# Autodesk Inventor assembly: Elevator HTD Iddler Pulley
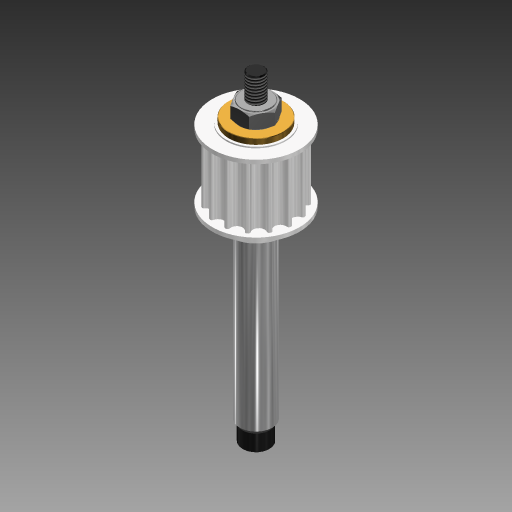
[picture p0: Inventor's stored thumbnail of the model, 512x512]
Saved by Autodesk Inventor 2023 (Build 270158030, 158C)
## iProperties
Created: 2023-02-09
Part Number: Elevator HTD Iddler Pulley
Document SubType Name: Assembly
Designer: Max Boord
Author: Max Boord
## Documents named in this file (11)
- D:\Collaborative Robots\COTS Parts\Elevators\Rev & WCP Elevator\Elevator HTD Iddler Pulley.iam
- D:\Collaborative Robots\COTS Parts\Power Transfer\Belts and Pullies\15T x 18mm Wide HTD 5mm Pulley (TTB-0058).ipt
- D:\Collaborative Robots\COTS Parts\Power Transfer\Bearings and Bushings\WCP 500 Hex Bushing.ipt
- D:\Collaborative Robots\COTS Parts\Hardware\Spacers\Spacers & Standoffs.ipt
- D:\Collaborative Robots\COTS Parts\Hardware\Fasteners\Washers.ipt
- D:\Collaborative Robots\COTS Parts\Hardware\Fasteners\Machine Screws.ipt
- D:\Collaborative Robots\COTS Parts\Hardware\Nuts and Threaded Blocks\Nuts\10-32 Pan Head Nylon locknut.ipt
- D:\Collaborative Robots\COTS Parts\Hardware\Nuts and Threaded Blocks\Nuts.ipt
- D:\Collaborative Robots\COTS Parts\Hardware\Fasteners\Machine Screws\10-32 UNFx3.5 Socket Head Cap Screw.ipt
- D:\Collaborative Robots\COTS Parts\Hardware\Spacers\Spacers & Standoffs\Aluminum Unthreaded Spacer (No. 10 x 3Lg x 0.375OD).ipt
- D:\Collaborative Robots\COTS Parts\Hardware\Fasteners\Washers\Washer 0.391ID 0.625OD 0.069Thick.ipt
## Components (7 placed, 6 different names)
1. 15T x 18mm Wide HTD 5mm Pulley (TTB-0058):1 — Insert:1, Insert:2
2. WCP 500 Hex Bushing:1 — Insert:2, Insert:11
3. WCP 500 Hex Bushing:2 — Insert:1, Insert:3
4. Aluminum Unthreaded Spacer (No. 10 x 3Lg x 0.375OD):1 — Insert:3, Insert:7, Mate:1
5. 10-32 UNFx3.5 Socket Head Cap Screw:1 — Mate:1, Insert:10
6. 10-32 Pan Head Nylon locknut:1 — Insert:7
7. Washer 0.391ID 0.625OD 0.069Thick:2 — Insert:10, Insert:11
## Relationships (7: Insert 6, Mate 1)
- Insert:1: 15T x 18mm Wide HTD 5mm Pulley (TTB-0058):1 ↔ WCP 500 Hex Bushing:2
- Insert:2: 15T x 18mm Wide HTD 5mm Pulley (TTB-0058):1 ↔ WCP 500 Hex Bushing:1
- Insert:3: WCP 500 Hex Bushing:2 ↔ Aluminum Unthreaded Spacer (No. 10 x 3Lg x 0.375OD):1
- Insert:7: Aluminum Unthreaded Spacer (No. 10 x 3Lg x 0.375OD):1 ↔ 10-32 Pan Head Nylon locknut:1
- Mate:1: Aluminum Unthreaded Spacer (No. 10 x 3Lg x 0.375OD):1 ↔ 10-32 UNFx3.5 Socket Head Cap Screw:1
- Insert:10 (50.8 mm): 10-32 UNFx3.5 Socket Head Cap Screw:1 ↔ Washer 0.391ID 0.625OD 0.069Thick:2
- Insert:11: WCP 500 Hex Bushing:1 ↔ Washer 0.391ID 0.625OD 0.069Thick:2
